# Autodesk Inventor assembly: Luz _1_
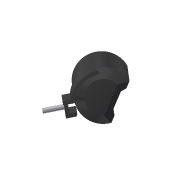
[picture p0: Inventor's stored thumbnail of the model, 180x180]
Saved by Autodesk Inventor 2019 (Build 230136000, 136)
## iProperties
Created: 2020-02-06
Part Number: Luz _1_
Document SubType Name: Assembly
Designer: Juan Carlos Botero
Author: Juan Carlos Botero
## Documents named in this file (4)
- D:\Drives\OneDrive\Carlos_2\02 TRABAJOS\MULTIPLO\Conveyor\ENSAMBLE\Luz _1_.iam
- D:\Drives\OneDrive\Carlos_2\02 TRABAJOS\MULTIPLO\Conveyor\ENSAMBLE\Tornillo reflector.ipt
- D:\Drives\OneDrive\Carlos_2\02 TRABAJOS\MULTIPLO\Conveyor\ENSAMBLE\Base reflector.ipt
- D:\Drives\OneDrive\Carlos_2\02 TRABAJOS\MULTIPLO\Conveyor\ENSAMBLE\Reflector.ipt
## Components (3 placed, 3 different names)
1. Tornillo reflector:1 — Rotational:1
2. Base reflector:1 — Tangent:1, Rotational:1, Flush:1, Angle:1
3. Reflector:1 — Tangent:1, Flush:1, Angle:1
## Relationships (4: Tangent 1, RevoluteJoint 1, Flush 1, Angle 1)
- Tangent:1: Base reflector:1 ↔ Reflector:1
- Rotational:1 [RevoluteJoint]: Tornillo reflector:1 ↔ Base reflector:1
- Flush:1 (30 mm): Base reflector:1 ↔ Reflector:1
- Angle:1 (45 deg): Base reflector:1 ↔ Reflector:1
